# Autodesk Inventor assembly: Stepper Motor NEMA 17
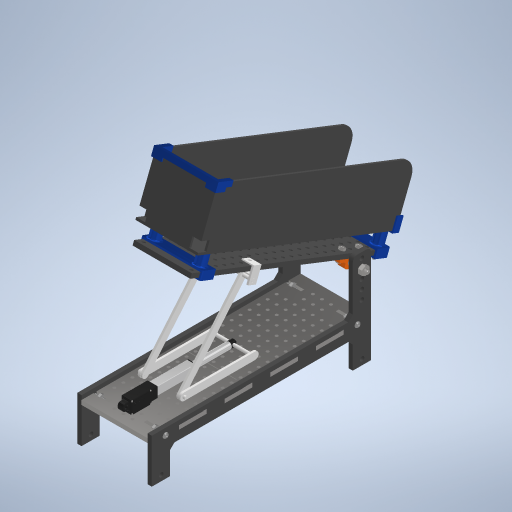
[picture p0: Inventor's stored thumbnail of the model, 512x512]
Saved by Autodesk Inventor 2024.1 (Build 281209000, 209)
## iProperties
Created: 2022-05-30
Part Number: Stepper Motor NEMA 17
Document SubType Name: Assembly
Designer: abdoo
Author: abdoo
## Documents named in this file (16)
- C:\Users\udayk\OneDrive\Desktop\Year 1\Engineer IP13\Project 3\My modelling\Stepper Motor NEMA 17.iam
- C:\Users\udayk\OneDrive\Desktop\Year 1\Engineer IP13\Project 3\Thurs-08 Modelling\2. Hopper Assembly\2. Hopper Assembly\Hopper.ipt
- C:\Users\udayk\OneDrive\Desktop\Year 1\Engineer IP13\Project 3\Thurs-08 Modelling\2. Hopper Assembly\2. Hopper Assembly\Connecting_Plate.iam
- C:\Users\udayk\OneDrive\Desktop\Year 1\Engineer IP13\Project 3\Thurs-08 Modelling\2. Hopper Assembly\2. Hopper Assembly\M4 Nut.ipt
- C:\Users\udayk\OneDrive\Desktop\Year 1\Engineer IP13\Project 3\Thurs-08 Modelling\2. Hopper Assembly\2. Hopper Assembly\Back-Clip.ipt
- C:\Users\udayk\OneDrive\Desktop\Year 1\Engineer IP13\Project 3\Thurs-08 Modelling\2. Hopper Assembly\2. Hopper Assembly\Corner Connector.ipt
- C:\Users\udayk\OneDrive\Desktop\Year 1\Engineer IP13\Project 3\Thurs-08 Modelling\2. Hopper Assembly\2. Hopper Assembly\Baseplate Assembley.iam
- C:\Users\udayk\OneDrive\Desktop\Year 1\Engineer IP13\Project 3\Thurs-08 Modelling\2. Hopper Assembly\2. Hopper Assembly\0.25 Inch x 4.5 inch Bolt.ipt
- C:\Users\udayk\OneDrive\Desktop\Year 1\Engineer IP13\Project 3\Thurs-08 Modelling\2. Hopper Assembly\2. Hopper Assembly\0.25 Inch Nut.ipt
- C:\Users\udayk\OneDrive\Desktop\Year 1\Engineer IP13\Project 3\Thurs-08 Modelling\2. Hopper Assembly\2. Hopper Assembly\M4 x 20mm Machine Screw.ipt
- C:\Users\udayk\OneDrive\Desktop\Year 1\Engineer IP13\Project 3\Thurs-08 Modelling\2. Hopper Assembly\2. Hopper Assembly\Front-Clip.ipt
- C:\Users\udayk\OneDrive\Desktop\Year 1\Engineer IP13\Project 3\Thurs-08 Modelling\2. Hopper Assembly\2. Hopper Assembly\98164A445_316 Stainless Steel Button Head Hex Drive Screw.ipt
- C:\Users\udayk\OneDrive\Desktop\Year 1\Engineer IP13\Project 3\Thurs-08 Modelling\2. Hopper Assembly\2. Hopper Assembly\Front.ipt
- C:\Users\udayk\OneDrive\Desktop\Year 1\Engineer IP13\Project 3\My modelling\final linear and linkage2.iam
- C:\Users\udayk\OneDrive\Desktop\Year 1\Engineer IP13\Project 3\My modelling\rodclamp1.ipt
- C:\Users\udayk\OneDrive\Desktop\Year 1\Engineer IP13\Project 3\My modelling\rod_for_clamp.ipt
## Components (24 placed, 15 different names)
1. Hopper:1 — Mate:1, Flush:1, Flush:2, Mate:20, Mate:21, Mate:22, Mate:84, Mate:85, Mate:86
2. Connecting_Plate:1 [sub-assembly] — Mate:1, Flush:1, Flush:2, Mate:23, Mate:24, Angle:1, Mate:27, Mate:28, Mate:73, Mate:74, Mate:75, Mate:88, Mate:89
3. Back-Clip:1 — Mate:23, Mate:24, Angle:1, Mate:77, Mate:79, Angle:3, Mate:83
4. Corner Connector:1 — Mate:20, Mate:21, Mate:22
5. Baseplate Assembley:1 [sub-assembly] — Mate:27, Mate:28, Mate:29, Mate:30, Mate:32, Mate:36, Mate:37, Mate:38, Mate:39, Mate:40, Mate:41, Mate:42, Mate:43, Mate:44, Mate:45, Mate:46, Mate:47, Mate:51, Mate:52, Mate:55, Mate:56, Mate:57, Mate:58, Mate:59, Mate:60, Mate:87, Angle:4, Flush:3
6. 0.25 Inch x 4.5 inch Bolt:1 — Mate:29, Mate:30, Mate:31
7. 0.25 Inch Nut:1 — Mate:31, Mate:32
8. M4 Nut:2 — Mate:36, Mate:37, Mate:38
9. M4 Nut:3 — Mate:39, Mate:44, Mate:45
10. M4 Nut:4 — Mate:40, Mate:43, Mate:46
11. M4 Nut:5 — Mate:41, Mate:42, Mate:47
12. M4 x 20mm Machine Screw:1 — Mate:51, Mate:52
13. M4 x 20mm Machine Screw:4 — Mate:55, Mate:56
14. M4 x 20mm Machine Screw:5 — Mate:57, Mate:58
15. M4 x 20mm Machine Screw:6 — Mate:59, Mate:60
16. Front-Clip:1 — Mate:73, Mate:74, Mate:75, Mate:76, Mate:78, Angle:2, Mate:81
17. M4 Nut:10 — Mate:80, Angle:2, Mate:81
18. 98164A445_316 Stainless Steel Button Head Hex Drive Screw:1 — Mate:76, Mate:78, Mate:80
19. 98164A445_316 Stainless Steel Button Head Hex Drive Screw:2 — Mate:77, Mate:79, Mate:82
20. M4 Nut:11 — Mate:82, Angle:3, Mate:83
21. Front:1 — Mate:84, Mate:85, Mate:86
22. final linear and linkage2:1 [sub-assembly] — Mate:87, Angle:4, Flush:3, Mate:91, Mate:92
23. rodclamp1:1 — Mate:88, Mate:89, Mate:90, Flush:4
24. rod_for_clamp:1 — Mate:90, Flush:4, Mate:91, Mate:92
## Relationships (60: Mate 52, Flush 4, Angle 4)
- Mate:1 (21 mm): Hopper:1 ↔ Connecting_Plate:1
- Flush:1 (3 mm): Hopper:1 ↔ Connecting_Plate:1
- Flush:2 (-3 mm): Hopper:1 ↔ Connecting_Plate:1
- Mate:20: Hopper:1 ↔ Corner Connector:1
- Mate:21: Hopper:1 ↔ Corner Connector:1
- Mate:22: Hopper:1 ↔ Corner Connector:1
- Mate:23: Connecting_Plate:1 ↔ Back-Clip:1
- Mate:24: Connecting_Plate:1 ↔ Back-Clip:1
- Angle:1 (0 deg): Connecting_Plate:1 ↔ Back-Clip:1
- Mate:27 (10 mm): Connecting_Plate:1 ↔ Baseplate Assembley:1
- Mate:28: Connecting_Plate:1 ↔ Baseplate Assembley:1
- Mate:29: Baseplate Assembley:1 ↔ 0.25 Inch x 4.5 inch Bolt:1
- Mate:30: Baseplate Assembley:1 ↔ 0.25 Inch x 4.5 inch Bolt:1
- Mate:31: 0.25 Inch x 4.5 inch Bolt:1 ↔ 0.25 Inch Nut:1
- Mate:32: Baseplate Assembley:1 ↔ 0.25 Inch Nut:1
- Mate:36 (0.5 mm): Baseplate Assembley:1 ↔ M4 Nut:2
- Mate:37 (0.5 mm): Baseplate Assembley:1 ↔ M4 Nut:2
- Mate:38 (0.5 mm): Baseplate Assembley:1 ↔ M4 Nut:2
- Mate:39 (0.5 mm): Baseplate Assembley:1 ↔ M4 Nut:3
- Mate:40 (0.5 mm): Baseplate Assembley:1 ↔ M4 Nut:4
- Mate:41: Baseplate Assembley:1 ↔ M4 Nut:5
- Mate:42 (0.5 mm): Baseplate Assembley:1 ↔ M4 Nut:5
- Mate:43 (0.5 mm): Baseplate Assembley:1 ↔ M4 Nut:4
- Mate:44 (0.5 mm): Baseplate Assembley:1 ↔ M4 Nut:3
- Mate:45 (0.5 mm): Baseplate Assembley:1 ↔ M4 Nut:3
- Mate:46 (0.5 mm): Baseplate Assembley:1 ↔ M4 Nut:4
- Mate:47 (0.5 mm): Baseplate Assembley:1 ↔ M4 Nut:5
- Mate:51: Baseplate Assembley:1 ↔ M4 x 20mm Machine Screw:1
- Mate:52: Baseplate Assembley:1 ↔ M4 x 20mm Machine Screw:1
- Mate:55: Baseplate Assembley:1 ↔ M4 x 20mm Machine Screw:4
- Mate:56: Baseplate Assembley:1 ↔ M4 x 20mm Machine Screw:4
- Mate:57: Baseplate Assembley:1 ↔ M4 x 20mm Machine Screw:5
- Mate:58: Baseplate Assembley:1 ↔ M4 x 20mm Machine Screw:5
- Mate:59: Baseplate Assembley:1 ↔ M4 x 20mm Machine Screw:6
- Mate:60: Baseplate Assembley:1 ↔ M4 x 20mm Machine Screw:6
- Mate:73 (0.2 mm): Connecting_Plate:1 ↔ Front-Clip:1
- Mate:74: Connecting_Plate:1 ↔ Front-Clip:1
- Mate:75: Connecting_Plate:1 ↔ Front-Clip:1
- Mate:76: Front-Clip:1 ↔ 98164A445_316 Stainless Steel Button Head Hex Drive Screw:1
- Mate:77: Back-Clip:1 ↔ 98164A445_316 Stainless Steel Button Head Hex Drive Screw:2
- Mate:78: Front-Clip:1 ↔ 98164A445_316 Stainless Steel Button Head Hex Drive Screw:1
- Mate:79: Back-Clip:1 ↔ 98164A445_316 Stainless Steel Button Head Hex Drive Screw:2
- Mate:80: M4 Nut:10 ↔ 98164A445_316 Stainless Steel Button Head Hex Drive Screw:1
- Angle:2 (0 deg): Front-Clip:1 ↔ M4 Nut:10
- Mate:81: Front-Clip:1 ↔ M4 Nut:10
- Mate:82: 98164A445_316 Stainless Steel Button Head Hex Drive Screw:2 ↔ M4 Nut:11
- Angle:3 (0 deg): Back-Clip:1 ↔ M4 Nut:11
- Mate:83: Back-Clip:1 ↔ M4 Nut:11
- Mate:84: Hopper:1 ↔ Front:1
- Mate:85: Hopper:1 ↔ Front:1
- Mate:86: Hopper:1 ↔ Front:1
- Mate:87: Baseplate Assembley:1 ↔ final linear and linkage2:1
- Angle:4 (-180 deg): Baseplate Assembley:1 ↔ final linear and linkage2:1
- Flush:3 (150 mm): Baseplate Assembley:1 ↔ final linear and linkage2:1
- Mate:88: Connecting_Plate:1 ↔ rodclamp1:1
- Mate:89: Connecting_Plate:1 ↔ rodclamp1:1
- Mate:90: rodclamp1:1 ↔ rod_for_clamp:1
- Flush:4: rodclamp1:1 ↔ rod_for_clamp:1
- Mate:91: final linear and linkage2:1 ↔ rod_for_clamp:1
- Mate:92: final linear and linkage2:1 ↔ rod_for_clamp:1
